# Autodesk Inventor assembly: Cup_Dispenser
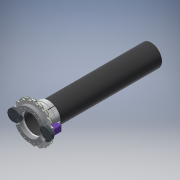
[picture p0: Inventor's stored thumbnail of the model, 180x180]
Saved by Autodesk Inventor 2016 (Build 200138000, 138)
## iProperties
Created: 2015-07-19
Part Number: Cup_Dispenser
Document SubType Name: Assembly
Designer: bastli
Author: bastli
## Documents named in this file (9)
- C:\Users\bastli\Documents\GitHub\BarBot\Conception\Mechanical\Cup_Dispenser_3\Cup_Dispenser.iam
- C:\Users\bastli\Documents\GitHub\BarBot\Conception\Mechanical\Cup_Dispenser_3\Fixture.ipt
- C:\Users\bastli\Documents\GitHub\BarBot\Conception\Mechanical\Cup_Dispenser_3\Transmission.ipt
- C:\Users\bastli\Documents\GitHub\BarBot\Conception\Mechanical\Cup_Dispenser_3\Nema 8.ipt
- C:\Users\bastli\Documents\GitHub\BarBot\Conception\Mechanical\Cup_Dispenser_3\Funnel_Adapter.ipt
- C:\Users\bastli\Documents\GitHub\BarBot\Conception\Mechanical\Cup_Dispenser_3\Hull.ipt
- C:\Users\bastli\Documents\GitHub\BarBot\Conception\Mechanical\Cup_Dispenser\Cup_Dispenser_Pipe.ipt
- C:\Users\bastli\Documents\GitHub\BarBot\Conception\Mechanical\Cup_Dispenser_3\Transmission_Mount_Tester.ipt
- C:\Users\bastli\Documents\GitHub\BarBot\Conception\Mechanical\Cup_Dispenser_3\Board_Shape.ipt
## Components (12 placed, 8 different names)
1. Fixture:1 — Rigid:1, Rigid:3, Flush:1, Rotational:3, Flush:2, Rigid:4, Flush:3, Rotational:4
2. Transmission:1 — Rotational:1
3. Nema 8:1 — Rigid:1, Rotational:1
4. Nema 8:2 — Rigid:3, Rotational:2
5. Transmission:2 — Rotational:2
6. Funnel_Adapter:1 — Flush:1
7. Funnel_Adapter:2 — Rotational:3
8. Hull:1 — Flush:2
9. Cup_Dispenser_Pipe:1 — Rigid:4
10. Transmission_Mount_Tester:1
11. Board_Shape:1 — Flush:3
12. Board_Shape:2 — Rotational:4
## Relationships (10: RevoluteJoint 4, WeldJoint 3, Flush 3)
- Rigid:1 [WeldJoint]: Fixture:1 ↔ Nema 8:1
- Rotational:1 [RevoluteJoint]: Transmission:1 ↔ Nema 8:1
- Rigid:3 [WeldJoint]: Fixture:1 ↔ Nema 8:2
- Rotational:2 [RevoluteJoint]: Nema 8:2 ↔ Transmission:2
- Flush:1: Fixture:1 ↔ Funnel_Adapter:1
- Rotational:3 [RevoluteJoint]: Fixture:1 ↔ Funnel_Adapter:2
- Flush:2: Fixture:1 ↔ Hull:1
- Rigid:4 [WeldJoint]: Fixture:1 ↔ Cup_Dispenser_Pipe:1
- Flush:3: Fixture:1 ↔ Board_Shape:1
- Rotational:4 [RevoluteJoint]: Fixture:1 ↔ Board_Shape:2
